# Autodesk Inventor assembly: Noodle Sucker
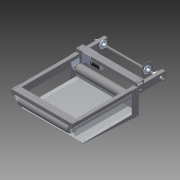
[picture p0: Inventor's stored thumbnail of the model, 180x180]
Saved by Autodesk Inventor 2015 SP1 (Build 190203100, 203)
## iProperties
Created: 2015-01-15
Part Number: Noodle Sucker
Document SubType Name: Assembly
Designer: 215152
Author: 215152
## Documents named in this file (24)
- C:\Users\Jarod\Documents\Westview\Robotics\FRC\2015\CAD\Robot\Noodle Sucker\Noodle Sucker.iam
- C:\Users\Jarod\Documents\Westview\Robotics\FRC\2015\CAD\Robot\Noodle Sucker\2x1.ipt
- C:\Users\Jarod\Documents\Westview\Robotics\FRC\2015\CAD\Robot\Noodle Sucker\Imported Components\Bearing Side Gusset\Bearing Side Gusset.ipt
- C:\Users\Jarod\Documents\Westview\Robotics\FRC\2015\CAD\Robot\Noodle Sucker\Imported Components\0.5 Hex Bearing\0.5 Hex Bearing.ipt
- C:\Users\Jarod\Documents\Westview\Robotics\FRC\2015\CAD\Robot\Noodle Sucker\2in roller front.ipt
- C:\Users\Jarod\Documents\Westview\Robotics\FRC\2015\CAD\Robot\Noodle Sucker\2in roller back.ipt
- C:\Users\Jarod\Documents\Westview\Robotics\FRC\2015\CAD\Robot\Noodle Sucker\roller hub.ipt
- C:\Users\Jarod\Documents\Westview\Robotics\FRC\2015\CAD\Robot\Noodle Sucker\0.5 hex shaft.ipt
- C:\Users\Jarod\Documents\Westview\Robotics\FRC\2015\CAD\Robot\Noodle Sucker\Imported Components\0.5 Hex Shaft Collar\0.5 Hex Shaft Collar.ipt
- C:\Users\Jarod\Documents\Westview\Robotics\FRC\2015\CAD\Robot\Noodle Sucker\Imported Components\0.5 Hex #25 Chain 16t Sprocket\0.5 Hex #25 Chain 16t Sprocket.ipt
- C:\Users\Jarod\Documents\Westview\Robotics\FRC\2015\CAD\Robot\Noodle Sucker\2x2 angle horizontal.ipt
- C:\Users\Jarod\Documents\Westview\Robotics\FRC\2015\CAD\Robot\Noodle Sucker\2x1 support horizontal.ipt
- C:\Users\Jarod\Documents\Westview\Robotics\FRC\2015\CAD\Robot\Noodle Sucker\Imported Components\2in horizontal gearbox mount\2in horizontal gearbox mount.ipt
- C:\Users\Jarod\Documents\Westview\Robotics\FRC\2015\CAD\Robot\Noodle Sucker\Imported Components\Versaplanetary Gearbox\Versaplanetary Gearbox.iam
- C:\Users\Jarod\Documents\Westview\Robotics\FRC\2015\CAD\Robot\Noodle Sucker\2x2 angle vertical right.ipt
- C:\Users\Jarod\Documents\Westview\Robotics\FRC\2015\CAD\Robot\Noodle Sucker\2x2 angle vertical left.ipt
- C:\Users\Jarod\Documents\Westview\Robotics\FRC\2015\CAD\Robot\Noodle Sucker\1x1 lengthwise right.ipt
- C:\Users\Jarod\Documents\Westview\Robotics\FRC\2015\CAD\Robot\Noodle Sucker\1x1 lengthwise left.ipt
- C:\Users\Jarod\Documents\Westview\Robotics\FRC\2015\CAD\Robot\Noodle Sucker\polycarb back.ipt
- C:\Users\Jarod\Documents\Westview\Robotics\FRC\2015\CAD\Robot\Noodle Sucker\polycarb bottom.ipt
- C:\Users\Jarod\Documents\Westview\Robotics\FRC\2015\CAD\Robot\Noodle Sucker\Imported Components\0.5 Hex Hub\0.5 Hex Hub.ipt
- C:\Users\Jarod\Documents\Westview\Robotics\FRC\2015\CAD\Robot\Noodle Sucker\0.5 hex shaft long.ipt
- C:\Users\Jarod\Documents\Westview\Robotics\FRC\2015\CAD\Robot\Noodle Sucker\Imported Components\Plate #25 Chain 48t Sprocket\Plate #25 Chain 48t Sprocket.ipt
- C:\Users\Jarod\Documents\Westview\Robotics\FRC\2015\CAD\Robot\Noodle Sucker\chain guard.ipt
## Components (54 placed, 23 different names)
1. 2x1:1 — Flush:1, Flush:2, Mate:1, Mate:2, Flush:5, Flush:6, Flush:8, Mate:43, Flush:14, Mate:44, Flush:15, Mate:68, Mate:85, Flush:26, Mate:89, Flush:27, Mate:92, Mate:95, Flush:29, Mate:98, Flush:31, Mate:106, Mate:112, Mate:113, Mate:114
2. 2x1:2 — Flush:1, Flush:2, Mate:3, Mate:4, Flush:3, Flush:4, Flush:7, Flush:17, Mate:51, Mate:70, Mate:93, Mate:94, Mate:99, Flush:30
3. 2x2 angle horizontal:1 — Mate:43, Flush:14, Mate:44, Flush:17
4. 2x1 support horizontal:1 — Flush:15, Mate:46, Flush:18, Mate:85, Flush:26
5. 2x2 angle vertical right:1 — Mate:68, Mate:72, Flush:23, Mate:80, Mate:81, Mate:89, Flush:27, Mate:90
6. 2x2 angle vertical left:1 — Mate:70, Mate:77, Flush:24, Mate:86, Mate:87, Mate:88, Mate:91
7. 1x1 lengthwise right:1 — Mate:72, Flush:23, Mate:82, Mate:83, Mate:90, Flush:28
8. 1x1 lengthwise left:1 — Mate:77, Flush:24, Mate:91
9. Bearing Side Gusset:1 — Mate:1, Flush:5, Flush:8, Mate:6, Mate:7, Mate:26
10. Bearing Side Gusset:2 — Mate:2, Flush:6, Mate:6, Mate:9, Mate:28
11. Bearing Side Gusset:3 — Mate:3, Flush:3, Mate:5, Flush:7, Mate:11, Mate:25
12. Bearing Side Gusset:4 — Mate:4, Flush:4, Mate:5, Mate:13, Mate:27
13. polycarb back:1 — Mate:80, Mate:81, Mate:82, Mate:84, Mate:86, Mate:88
14. polycarb bottom:1 — Mate:83, Mate:84, Mate:87, Flush:28
15. 2in roller front:1 — Mate:15, Mate:17, Flush:9, Mate:19, Flush:11
16. 2in roller back:1 — Mate:16, Mate:18, Flush:10, Mate:20, Flush:12
17. roller hub:1 — Mate:17, Flush:9, Mate:60
18. roller hub:2 — Mate:18, Flush:10, Mate:58
19. roller hub:3 — Mate:19, Flush:11, Mate:61
20. roller hub:4 — Mate:20, Flush:12, Mate:62
21. 2in horizontal gearbox mount:1 — Mate:46, Flush:18, Mate:47, Mate:48, Mate:49, Mate:51
22. Versaplanetary Gearbox:1 [sub-assembly] — Mate:47, Mate:48, Mate:49, Mate:50, Mate:52
23. 0.5 Hex Hub:1 — Mate:92, Mate:95, Mate:96, Mate:97, Mate:107
24. 0.5 Hex Hub:2 — Mate:93, Mate:94
25. 0.5 Hex Hub:3 — Mate:104, Mate:105, Mate:107, Mate:108, Mate:109, Mate:110, Mate:111
26. 0.5 hex shaft:1 — Mate:21, Mate:22, Flush:19
27. 0.5 hex shaft:2 — Mate:23, Mate:24, Flush:20
28. 0.5 hex shaft long:1 — Mate:96, Mate:97, Flush:29
29. 0.5 Hex Bearing:1 — Mate:7, Mate:15, Mate:21, Mate:22, Mate:26, Mate:32, Mate:35, Mate:37, Mate:38, Mate:54
30. 0.5 Hex Bearing:2 — Mate:9, Mate:16, Mate:23, Mate:24, Mate:28, Mate:31, Mate:36, Mate:39, Mate:40, Mate:56
31. 0.5 Hex Bearing:3 — Mate:11, Mate:25, Mate:29, Mate:33, Mate:53
32. 0.5 Hex Bearing:4 — Mate:13, Mate:27, Mate:30, Mate:34, Mate:41, Mate:42, Mate:55, Mate:63
33. 0.5 Hex Bearing:5 — Mate:98, Mate:101, Mate:102, Flush:31
34. 0.5 Hex Bearing:6 — Mate:99, Mate:100, Mate:103, Flush:30
35. 0.5 Hex Shaft Collar:1 — Mate:32, Mate:35, Flush:19
36. 0.5 Hex Shaft Collar:2 — Mate:31, Mate:36, Flush:20
37. 0.5 Hex Shaft Collar:3 — Mate:29, Mate:33
38. 0.5 Hex Shaft Collar:4 — Mate:30, Mate:34
39. 0.5 Hex Shaft Collar:5 — Mate:54, Mate:59, Mate:60
40. 0.5 Hex Shaft Collar:6 — Mate:56, Mate:57, Mate:58
41. 0.5 Hex Shaft Collar:7 — Mate:53, Mate:61
42. 0.5 Hex Shaft Collar:8 — Mate:55, Mate:62
43. 0.5 Hex Shaft Collar:9 — Mate:63, Mate:64
44. 0.5 Hex Shaft Collar:10 — Mate:65, Mate:66
45. 0.5 Hex Shaft Collar:11 — Mate:101, Mate:102
46. 0.5 Hex Shaft Collar:12 — Mate:100, Mate:103
47. 0.5 Hex Shaft Collar:13 — Mate:108, Mate:110
48. 0.5 Hex Shaft Collar:14 — Mate:109, Mate:111
49. 0.5 Hex #25 Chain 16t Sprocket:1 — Mate:37, Mate:38, Mate:59
50. 0.5 Hex #25 Chain 16t Sprocket:2 — Mate:39, Mate:40, Mate:57
51. 0.5 Hex #25 Chain 16t Sprocket:3 — Mate:41, Mate:42, Mate:64
52. 0.5 Hex #25 Chain 16t Sprocket:4 — Mate:50, Mate:52, Mate:65, Mate:66
53. Plate #25 Chain 48t Sprocket:1 — Mate:104, Mate:105, Mate:106
54. chain guard:1 — Mate:112, Mate:113, Mate:114
## Relationships (126: Mate 100, Flush 26)
- Flush:1: 2x1:1 ↔ 2x1:2
- Flush:2: 2x1:1 ↔ 2x1:2
- Mate:1: 2x1:1 ↔ Bearing Side Gusset:1
- Mate:2: 2x1:1 ↔ Bearing Side Gusset:2
- Mate:3: 2x1:2 ↔ Bearing Side Gusset:3
- Mate:4: 2x1:2 ↔ Bearing Side Gusset:4
- Flush:3 (25.4 mm): 2x1:2 ↔ Bearing Side Gusset:3
- Flush:4 (25.4 mm): 2x1:2 ↔ Bearing Side Gusset:4
- Flush:5 (25.4 mm): 2x1:1 ↔ Bearing Side Gusset:1
- Flush:6 (25.4 mm): 2x1:1 ↔ Bearing Side Gusset:2
- Mate:5 (368.3 mm): Bearing Side Gusset:3 ↔ Bearing Side Gusset:4
- Flush:7: 2x1:2 ↔ Bearing Side Gusset:3
- Flush:8: 2x1:1 ↔ Bearing Side Gusset:1
- Mate:6 (368.3 mm): Bearing Side Gusset:1 ↔ Bearing Side Gusset:2
- Mate:7: Bearing Side Gusset:1 ↔ 0.5 Hex Bearing:1
- Mate:9: Bearing Side Gusset:2 ↔ 0.5 Hex Bearing:2
- Mate:11: Bearing Side Gusset:3 ↔ 0.5 Hex Bearing:3
- Mate:13: Bearing Side Gusset:4 ↔ 0.5 Hex Bearing:4
- Mate:15: 2in roller front:1 ↔ 0.5 Hex Bearing:1
- Mate:16: 2in roller back:1 ↔ 0.5 Hex Bearing:2
- Mate:17: 2in roller front:1 ↔ roller hub:1
- Flush:9: 2in roller front:1 ↔ roller hub:1
- Mate:18: 2in roller back:1 ↔ roller hub:2
- Flush:10: 2in roller back:1 ↔ roller hub:2
- Mate:19: 2in roller front:1 ↔ roller hub:3
- Flush:11: 2in roller front:1 ↔ roller hub:3
- Mate:20: 2in roller back:1 ↔ roller hub:4
- Flush:12: 2in roller back:1 ↔ roller hub:4
- Mate:21: 0.5 hex shaft:1 ↔ 0.5 Hex Bearing:1
- Mate:22: 0.5 hex shaft:1 ↔ 0.5 Hex Bearing:1
- Mate:23: 0.5 hex shaft:2 ↔ 0.5 Hex Bearing:2
- Mate:24: 0.5 hex shaft:2 ↔ 0.5 Hex Bearing:2
- Mate:25: Bearing Side Gusset:3 ↔ 0.5 Hex Bearing:3
- Mate:26: Bearing Side Gusset:1 ↔ 0.5 Hex Bearing:1
- Mate:27: Bearing Side Gusset:4 ↔ 0.5 Hex Bearing:4
- Mate:28: Bearing Side Gusset:2 ↔ 0.5 Hex Bearing:2
- Mate:29: 0.5 Hex Bearing:3 ↔ 0.5 Hex Shaft Collar:3
- Mate:30: 0.5 Hex Bearing:4 ↔ 0.5 Hex Shaft Collar:4
- Mate:31: 0.5 Hex Bearing:2 ↔ 0.5 Hex Shaft Collar:2
- Mate:32: 0.5 Hex Bearing:1 ↔ 0.5 Hex Shaft Collar:1
- Mate:33: 0.5 Hex Bearing:3 ↔ 0.5 Hex Shaft Collar:3
- Mate:34: 0.5 Hex Bearing:4 ↔ 0.5 Hex Shaft Collar:4
- Mate:35: 0.5 Hex Bearing:1 ↔ 0.5 Hex Shaft Collar:1
- Mate:36: 0.5 Hex Bearing:2 ↔ 0.5 Hex Shaft Collar:2
- Mate:37: 0.5 Hex Bearing:1 ↔ 0.5 Hex #25 Chain 16t Sprocket:1
- Mate:38: 0.5 Hex Bearing:1 ↔ 0.5 Hex #25 Chain 16t Sprocket:1
- Mate:39: 0.5 Hex Bearing:2 ↔ 0.5 Hex #25 Chain 16t Sprocket:2
- Mate:40: 0.5 Hex Bearing:2 ↔ 0.5 Hex #25 Chain 16t Sprocket:2
- Mate:41: 0.5 Hex Bearing:4 ↔ 0.5 Hex #25 Chain 16t Sprocket:3
- Mate:42: 0.5 Hex Bearing:4 ↔ 0.5 Hex #25 Chain 16t Sprocket:3
- Mate:43: 2x1:1 ↔ 2x2 angle horizontal:1
- Flush:14: 2x1:1 ↔ 2x2 angle horizontal:1
- Mate:44: 2x1:1 ↔ 2x2 angle horizontal:1
- Flush:15: 2x1:1 ↔ 2x1 support horizontal:1
- Flush:17: 2x1:2 ↔ 2x2 angle horizontal:1
- Mate:46: 2x1 support horizontal:1 ↔ 2in horizontal gearbox mount:1
- Flush:18: 2x1 support horizontal:1 ↔ 2in horizontal gearbox mount:1
- Mate:47: 2in horizontal gearbox mount:1 ↔ Versaplanetary Gearbox:1
- Mate:48: 2in horizontal gearbox mount:1 ↔ Versaplanetary Gearbox:1
- Mate:49: 2in horizontal gearbox mount:1 ↔ Versaplanetary Gearbox:1
- Mate:50: Versaplanetary Gearbox:1 ↔ 0.5 Hex #25 Chain 16t Sprocket:4
- Mate:51 (19.05 mm): 2x1:2 ↔ 2in horizontal gearbox mount:1
- Mate:52: Versaplanetary Gearbox:1 ↔ 0.5 Hex #25 Chain 16t Sprocket:4
- Mate:53: 0.5 Hex Bearing:3 ↔ 0.5 Hex Shaft Collar:7
- Mate:54: 0.5 Hex Bearing:1 ↔ 0.5 Hex Shaft Collar:5
- Mate:55: 0.5 Hex Bearing:4 ↔ 0.5 Hex Shaft Collar:8
- Mate:56: 0.5 Hex Bearing:2 ↔ 0.5 Hex Shaft Collar:6
- Mate:57: 0.5 Hex Shaft Collar:6 ↔ 0.5 Hex #25 Chain 16t Sprocket:2
- Mate:58: roller hub:2 ↔ 0.5 Hex Shaft Collar:6
- Mate:59: 0.5 Hex Shaft Collar:5 ↔ 0.5 Hex #25 Chain 16t Sprocket:1
- Mate:60: roller hub:1 ↔ 0.5 Hex Shaft Collar:5
- Mate:61: roller hub:3 ↔ 0.5 Hex Shaft Collar:7
- Mate:62: roller hub:4 ↔ 0.5 Hex Shaft Collar:8
- Mate:63: 0.5 Hex Bearing:4 ↔ 0.5 Hex Shaft Collar:9
- Mate:64: 0.5 Hex Shaft Collar:9 ↔ 0.5 Hex #25 Chain 16t Sprocket:3
- Mate:65: 0.5 Hex Shaft Collar:10 ↔ 0.5 Hex #25 Chain 16t Sprocket:4
- Mate:66: 0.5 Hex Shaft Collar:10 ↔ 0.5 Hex #25 Chain 16t Sprocket:4
- Flush:19 (-6.35 mm): 0.5 hex shaft:1 ↔ 0.5 Hex Shaft Collar:1
- Flush:20 (-6.35 mm): 0.5 hex shaft:2 ↔ 0.5 Hex Shaft Collar:2
- Mate:68: 2x1:1 ↔ 2x2 angle vertical right:1
- Mate:70: 2x1:2 ↔ 2x2 angle vertical left:1
- Mate:72: 2x2 angle vertical right:1 ↔ 1x1 lengthwise right:1
- Flush:23: 2x2 angle vertical right:1 ↔ 1x1 lengthwise right:1
- Mate:77: 2x2 angle vertical left:1 ↔ 1x1 lengthwise left:1
- Flush:24: 2x2 angle vertical left:1 ↔ 1x1 lengthwise left:1
- Mate:80: 2x2 angle vertical right:1 ↔ polycarb back:1
- Mate:81: 2x2 angle vertical right:1 ↔ polycarb back:1
- Mate:82: 1x1 lengthwise right:1 ↔ polycarb back:1
- Mate:83: 1x1 lengthwise right:1 ↔ polycarb bottom:1
- Mate:84: polycarb back:1 ↔ polycarb bottom:1
- Mate:85: 2x1:1 ↔ 2x1 support horizontal:1
- Flush:26 (495.3 mm): 2x1:1 ↔ 2x1 support horizontal:1
- Mate:86: 2x2 angle vertical left:1 ↔ polycarb back:1
- Mate:87: 2x2 angle vertical left:1 ↔ polycarb bottom:1
- Mate:88: 2x2 angle vertical left:1 ↔ polycarb back:1
- Mate:89: 2x1:1 ↔ 2x2 angle vertical right:1
- Flush:27 (450.85 mm): 2x1:1 ↔ 2x2 angle vertical right:1
- Mate:90: 2x2 angle vertical right:1 ↔ 1x1 lengthwise right:1
- Mate:91: 2x2 angle vertical left:1 ↔ 1x1 lengthwise left:1
- Flush:28: 1x1 lengthwise right:1 ↔ polycarb bottom:1
- Mate:92: 2x1:1 ↔ 0.5 Hex Hub:1
- Mate:93: 2x1:2 ↔ 0.5 Hex Hub:2
- Mate:94: 2x1:2 ↔ 0.5 Hex Hub:2
- Mate:95: 2x1:1 ↔ 0.5 Hex Hub:1
- Mate:96: 0.5 Hex Hub:1 ↔ 0.5 hex shaft long:1
- Mate:97: 0.5 Hex Hub:1 ↔ 0.5 hex shaft long:1
- Flush:29 (-31.75 mm): 2x1:1 ↔ 0.5 hex shaft long:1
- Mate:98: 2x1:1 ↔ 0.5 Hex Bearing:5
- Mate:99: 2x1:2 ↔ 0.5 Hex Bearing:6
- Mate:100: 0.5 Hex Bearing:6 ↔ 0.5 Hex Shaft Collar:12
- Mate:101: 0.5 Hex Bearing:5 ↔ 0.5 Hex Shaft Collar:11
- Mate:102: 0.5 Hex Bearing:5 ↔ 0.5 Hex Shaft Collar:11
- Mate:103: 0.5 Hex Bearing:6 ↔ 0.5 Hex Shaft Collar:12
- Flush:30 (-10.3188 mm): 2x1:2 ↔ 0.5 Hex Bearing:6
- Flush:31 (-10.3188 mm): 2x1:1 ↔ 0.5 Hex Bearing:5
- Mate:104: 0.5 Hex Hub:3 ↔ Plate #25 Chain 48t Sprocket:1
- Mate:105: 0.5 Hex Hub:3 ↔ Plate #25 Chain 48t Sprocket:1
- Mate:106 (79.375 mm): 2x1:1 ↔ Plate #25 Chain 48t Sprocket:1
- Mate:107: 0.5 Hex Hub:1 ↔ 0.5 Hex Hub:3
- Mate:108: 0.5 Hex Hub:3 ↔ 0.5 Hex Shaft Collar:13
- Mate:109: 0.5 Hex Hub:3 ↔ 0.5 Hex Shaft Collar:14
- Mate:110: 0.5 Hex Hub:3 ↔ 0.5 Hex Shaft Collar:13
- Mate:111: 0.5 Hex Hub:3 ↔ 0.5 Hex Shaft Collar:14
- Mate:112: 2x1:1 ↔ chain guard:1
- Mate:113: 2x1:1 ↔ chain guard:1
- Mate:114: 2x1:1 ↔ chain guard:1
